# Autodesk Inventor assembly: PMax6
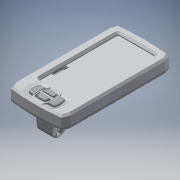
[picture p0: Inventor's stored thumbnail of the model, 180x180]
Saved by Autodesk Inventor 2018 (Build 220112000, 112)
## iProperties
Created: 2019-05-29
Part Number: PMax6
Document SubType Name: Assembly
Designer: Ash
Author: Ash
## Documents named in this file (6)
- C:\Autodesk\Skills 2019 Nationals\Competition\PMDay2\PMax6.iam
- C:\Autodesk\Skills 2019 Nationals\Competition\PMDay2\#2-KEYPAD.ipt
- C:\Autodesk\Skills 2019 Nationals\Competition\PMDay2\#4-GASKET(PMAX6).ipt
- C:\Autodesk\Skills 2019 Nationals\Competition\PMDay2\#5-BACK_COVER(PMAX6).ipt
- C:\Autodesk\Skills 2019 Nationals\Competition\PMDay1\Display_Plate2.ipt
- C:\Autodesk\Skills 2019 Nationals\Competition\PMDay1\Front_Cover2.ipt
## Components (5 placed, 5 different names)
1. #2-KEYPAD:1 — Mate:6, Mate:7, Mate:8, Mate:9, Mate:11
2. Display_Plate2:1 — Mate:7, Mate:10, Mate:11
3. Front_Cover2:1 — Mate:6, Mate:8, Mate:9, Mate:10, Mate:23, Mate:24, Mate:25
4. #5-BACK_COVER(PMAX6):1 — Mate:12, Mate:13, Mate:14, Mate:23, Mate:24, Mate:25
5. #4-GASKET(PMAX6):1 — Mate:12, Mate:13, Mate:14
## Relationships (12: Mate 12)
- Mate:6 (6.35 mm): #2-KEYPAD:1 ↔ Front_Cover2:1
- Mate:7: #2-KEYPAD:1 ↔ Display_Plate2:1
- Mate:8: #2-KEYPAD:1 ↔ Front_Cover2:1
- Mate:9 (46.7868 mm): #2-KEYPAD:1 ↔ Front_Cover2:1
- Mate:10: Display_Plate2:1 ↔ Front_Cover2:1
- Mate:11: #2-KEYPAD:1 ↔ Display_Plate2:1
- Mate:12: #5-BACK_COVER(PMAX6):1 ↔ #4-GASKET(PMAX6):1
- Mate:13: #5-BACK_COVER(PMAX6):1 ↔ #4-GASKET(PMAX6):1
- Mate:14: #5-BACK_COVER(PMAX6):1 ↔ #4-GASKET(PMAX6):1
- Mate:23: Front_Cover2:1 ↔ #5-BACK_COVER(PMAX6):1
- Mate:24: Front_Cover2:1 ↔ #5-BACK_COVER(PMAX6):1
- Mate:25: Front_Cover2:1 ↔ #5-BACK_COVER(PMAX6):1
